# Autodesk Inventor assembly: ProbeHead - Assembly
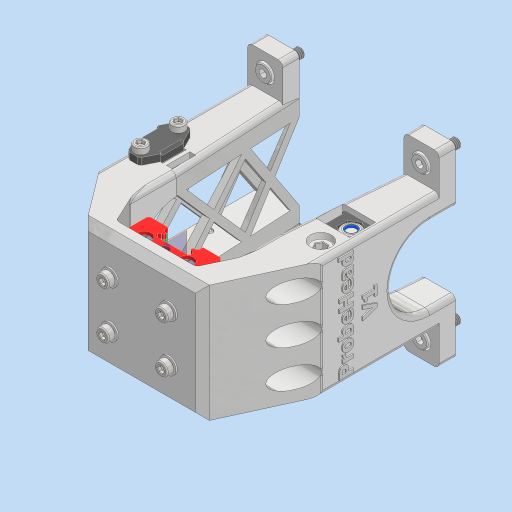
[picture p0: Inventor's stored thumbnail of the model, 512x512]
Saved by Autodesk Inventor 2023.2 (Build 272271000, 271)
## iProperties
Created: 2024-02-09
Part Number: ProbeHead - Assembly
Document SubType Name: Assembly
Designer: Nils Bade
Author: Nils Bade
## Documents named in this file (11)
- C:\Users\nilsb\Documents\Inventor\Projektarbeit-Bade\RatRig_modified\ProbeHead\ProbeHead - Assembly.iam
- C:\Users\nilsb\Documents\Inventor\Projektarbeit-Bade\RatRig_Standards\core_xy_belt_grabber v2.ipt
- C:\Users\nilsb\Documents\Inventor\Projektarbeit-Bade\RatRig_modified\MGN15 Linear-Rail-Block.ipt
- C:\Users\nilsb\Documents\Inventor\Projektarbeit-Bade\RatRig_modified\ProbeHead\ProbeHead-Arms V1.ipt
- C:\Users\nilsb\Documents\Inventor\Projektarbeit-Bade\RatRig_Standards\face_belt_grabber v2.ipt
- C:\Users\nilsb\Documents\Inventor\Projektarbeit-Bade\Schrauben\Cap Head Screw M3x12 v2.ipt
- C:\Users\nilsb\Documents\Inventor\Projektarbeit-Bade\RatRig_Standards\Hex Nut - M3 v2.ipt
- C:\Users\nilsb\Documents\Inventor\Projektarbeit-Bade\Schrauben\Cap Head Screw M5x40 v2.ipt
- C:\Users\nilsb\Documents\Inventor\Projektarbeit-Bade\RatRig_Standards\Hex Locking Nut - M5 v2.ipt
- C:\Users\nilsb\Documents\Inventor\Projektarbeit-Bade\Schrauben\Cap Head Screw M4x12 - DIN912.ipt
- C:\Users\nilsb\Documents\Inventor\Projektarbeit-Bade\Schrauben\Washer Simple M3 - DIN6902.ipt
## Components (30 placed, 10 different names)
1. ProbeHead-Arms V1:1 — Passend:1, Passend:2, Passend:3, Passend:4, Winkel:1, Winkel:2, Passend:5, Fluchtend:1, Fluchtend:2, Passend:6, Passend:8, Passend:9, Passend:11, Winkel:3, Winkel:6, Passend:24, Passend:25, Passend:26, Passend:27, Passend:28, Passend:29, Passend:30, Passend:31, Passend:36, Passend:37, Passend:38, Passend:39, Passend:40, Passend:41, Passend:42, Passend:43, Passend:44, Passend:45, Passend:46, Passend:47, Passend:48, Passend:49, Passend:50, Passend:51, Passend:52, Passend:53, Passend:54, Passend:55, Passend:60, Passend:61, Winkel:9, Winkel:10
2. core_xy_belt_grabber v2:1 — Winkel:2, Passend:5, Fluchtend:1, Winkel:7, Passend:35
3. core_xy_belt_grabber v2:2 — Passend:4, Winkel:1, Fluchtend:2, Passend:32, Passend:33, Winkel:8
4. MGN15 Linear-Rail-Block:1 — Passend:1, Passend:2, Passend:3
5. face_belt_grabber v2:1 — Passend:9, Passend:11, Passend:16, Passend:17, Passend:18, Passend:19
6. face_belt_grabber v2:2 — Passend:6, Passend:8, Passend:12, Passend:13, Passend:14, Passend:15
7. Cap Head Screw M3x12 v2:1 — Passend:16, Passend:18, Passend:20
8. Cap Head Screw M3x12 v2:2 — Passend:17, Passend:19, Passend:21, Passend:61
9. Cap Head Screw M3x12 v2:3 — Passend:12, Passend:14, Passend:22
10. Cap Head Screw M3x12 v2:4 — Passend:13, Passend:15, Passend:23, Passend:60
11. Hex Nut - M3 v2:1 — Passend:20, Winkel:3, Passend:26
12. Hex Nut - M3 v2:2 — Passend:23, Passend:25, Winkel:9
13. Hex Nut - M3 v2:3 — Passend:22, Winkel:6, Passend:24
14. Hex Nut - M3 v2:4 — Passend:21, Passend:27, Winkel:10
15. Cap Head Screw M5x40 v2:1 — Passend:29, Passend:30, Passend:34
16. Cap Head Screw M5x40 v2:2 — Passend:28, Passend:31
17. Hex Locking Nut - M5 v2:1 — Passend:32, Passend:33, Winkel:8
18. Hex Locking Nut - M5 v2:2 — Passend:34, Winkel:7, Passend:35
19. Cap Head Screw M4x12 - DIN912:1 — Passend:36, Passend:40
20. Cap Head Screw M4x12 - DIN912:2 — Passend:37, Passend:41
21. Cap Head Screw M4x12 - DIN912:3 — Passend:39, Passend:43
22. Cap Head Screw M4x12 - DIN912:4 — Passend:38, Passend:42
23. Washer Simple M3 - DIN6902:1 — Passend:44, Passend:50, Passend:59
24. Washer Simple M3 - DIN6902:2 — Passend:45, Passend:49, Passend:56
25. Washer Simple M3 - DIN6902:3 — Passend:46, Passend:51, Passend:58
26. Washer Simple M3 - DIN6902:4 — Passend:47, Passend:48, Passend:57
27. Cap Head Screw M3x12 v2:5 — Passend:52, Passend:59
28. Cap Head Screw M3x12 v2:6 — Passend:53, Passend:58
29. Cap Head Screw M3x12 v2:7 — Passend:54, Passend:56
30. Cap Head Screw M3x12 v2:8 — Passend:55, Passend:57
## Relationships (69: Mate 59, Angle 8, Flush 2)
- Passend:1 [Mate]: ProbeHead-Arms V1:1 ↔ MGN15 Linear-Rail-Block:1
- Passend:2 [Mate]: ProbeHead-Arms V1:1 ↔ MGN15 Linear-Rail-Block:1
- Passend:3 [Mate]: ProbeHead-Arms V1:1 ↔ MGN15 Linear-Rail-Block:1
- Passend:4 [Mate]: ProbeHead-Arms V1:1 ↔ core_xy_belt_grabber v2:2
- Winkel:1 [Angle] (0 deg): ProbeHead-Arms V1:1 ↔ core_xy_belt_grabber v2:2
- Winkel:2 [Angle] (0 deg): ProbeHead-Arms V1:1 ↔ core_xy_belt_grabber v2:1
- Passend:5 [Mate]: ProbeHead-Arms V1:1 ↔ core_xy_belt_grabber v2:1
- Fluchtend:1 [Flush] (2 mm): ProbeHead-Arms V1:1 ↔ core_xy_belt_grabber v2:1
- Fluchtend:2 [Flush] (2 mm): ProbeHead-Arms V1:1 ↔ core_xy_belt_grabber v2:2
- Passend:6 [Mate]: ProbeHead-Arms V1:1 ↔ face_belt_grabber v2:2
- Passend:8 [Mate]: ProbeHead-Arms V1:1 ↔ face_belt_grabber v2:2
- Passend:9 [Mate]: ProbeHead-Arms V1:1 ↔ face_belt_grabber v2:1
- Passend:11 [Mate]: ProbeHead-Arms V1:1 ↔ face_belt_grabber v2:1
- Passend:12 [Mate]: face_belt_grabber v2:2 ↔ Cap Head Screw M3x12 v2:3
- Passend:13 [Mate]: face_belt_grabber v2:2 ↔ Cap Head Screw M3x12 v2:4
- Passend:14 [Mate]: face_belt_grabber v2:2 ↔ Cap Head Screw M3x12 v2:3
- Passend:15 [Mate]: face_belt_grabber v2:2 ↔ Cap Head Screw M3x12 v2:4
- Passend:16 [Mate]: face_belt_grabber v2:1 ↔ Cap Head Screw M3x12 v2:1
- Passend:17 [Mate]: face_belt_grabber v2:1 ↔ Cap Head Screw M3x12 v2:2
- Passend:18 [Mate]: face_belt_grabber v2:1 ↔ Cap Head Screw M3x12 v2:1
- Passend:19 [Mate]: face_belt_grabber v2:1 ↔ Cap Head Screw M3x12 v2:2
- Passend:20 [Mate]: Cap Head Screw M3x12 v2:1 ↔ Hex Nut - M3 v2:1
- Passend:21 [Mate]: Cap Head Screw M3x12 v2:2 ↔ Hex Nut - M3 v2:4
- Passend:22 [Mate]: Cap Head Screw M3x12 v2:3 ↔ Hex Nut - M3 v2:3
- Passend:23 [Mate]: Cap Head Screw M3x12 v2:4 ↔ Hex Nut - M3 v2:2
- Winkel:3 [Angle] (0 deg): ProbeHead-Arms V1:1 ↔ Hex Nut - M3 v2:1
- Winkel:6 [Angle] (0 deg): ProbeHead-Arms V1:1 ↔ Hex Nut - M3 v2:3
- Passend:24 [Mate]: ProbeHead-Arms V1:1 ↔ Hex Nut - M3 v2:3
- Passend:25 [Mate]: ProbeHead-Arms V1:1 ↔ Hex Nut - M3 v2:2
- Passend:26 [Mate]: ProbeHead-Arms V1:1 ↔ Hex Nut - M3 v2:1
- Passend:27 [Mate]: ProbeHead-Arms V1:1 ↔ Hex Nut - M3 v2:4
- Passend:28 [Mate]: ProbeHead-Arms V1:1 ↔ Cap Head Screw M5x40 v2:2
- Passend:29 [Mate]: ProbeHead-Arms V1:1 ↔ Cap Head Screw M5x40 v2:1
- Passend:30 [Mate]: ProbeHead-Arms V1:1 ↔ Cap Head Screw M5x40 v2:1
- Passend:31 [Mate]: ProbeHead-Arms V1:1 ↔ Cap Head Screw M5x40 v2:2
- Passend:32 [Mate]: core_xy_belt_grabber v2:2 ↔ Hex Locking Nut - M5 v2:1
- Passend:33 [Mate]: core_xy_belt_grabber v2:2 ↔ Hex Locking Nut - M5 v2:1
- Passend:34 [Mate]: Cap Head Screw M5x40 v2:1 ↔ Hex Locking Nut - M5 v2:2
- Winkel:7 [Angle] (0 deg): core_xy_belt_grabber v2:1 ↔ Hex Locking Nut - M5 v2:2
- Passend:35 [Mate]: core_xy_belt_grabber v2:1 ↔ Hex Locking Nut - M5 v2:2
- Winkel:8 [Angle] (0 deg): core_xy_belt_grabber v2:2 ↔ Hex Locking Nut - M5 v2:1
- Passend:36 [Mate]: ProbeHead-Arms V1:1 ↔ Cap Head Screw M4x12 - DIN912:1
- Passend:37 [Mate]: ProbeHead-Arms V1:1 ↔ Cap Head Screw M4x12 - DIN912:2
- Passend:38 [Mate]: ProbeHead-Arms V1:1 ↔ Cap Head Screw M4x12 - DIN912:4
- Passend:39 [Mate]: ProbeHead-Arms V1:1 ↔ Cap Head Screw M4x12 - DIN912:3
- Passend:40 [Mate]: ProbeHead-Arms V1:1 ↔ Cap Head Screw M4x12 - DIN912:1
- Passend:41 [Mate]: ProbeHead-Arms V1:1 ↔ Cap Head Screw M4x12 - DIN912:2
- Passend:42 [Mate]: ProbeHead-Arms V1:1 ↔ Cap Head Screw M4x12 - DIN912:4
- Passend:43 [Mate]: ProbeHead-Arms V1:1 ↔ Cap Head Screw M4x12 - DIN912:3
- Passend:44 [Mate]: ProbeHead-Arms V1:1 ↔ Washer Simple M3 - DIN6902:1
- Passend:45 [Mate]: ProbeHead-Arms V1:1 ↔ Washer Simple M3 - DIN6902:2
- Passend:46 [Mate]: ProbeHead-Arms V1:1 ↔ Washer Simple M3 - DIN6902:3
- Passend:47 [Mate]: ProbeHead-Arms V1:1 ↔ Washer Simple M3 - DIN6902:4
- Passend:48 [Mate]: ProbeHead-Arms V1:1 ↔ Washer Simple M3 - DIN6902:4
- Passend:49 [Mate]: ProbeHead-Arms V1:1 ↔ Washer Simple M3 - DIN6902:2
- Passend:50 [Mate]: ProbeHead-Arms V1:1 ↔ Washer Simple M3 - DIN6902:1
- Passend:51 [Mate]: ProbeHead-Arms V1:1 ↔ Washer Simple M3 - DIN6902:3
- Passend:52 [Mate]: ProbeHead-Arms V1:1 ↔ Cap Head Screw M3x12 v2:5
- Passend:53 [Mate]: ProbeHead-Arms V1:1 ↔ Cap Head Screw M3x12 v2:6
- Passend:54 [Mate]: ProbeHead-Arms V1:1 ↔ Cap Head Screw M3x12 v2:7
- Passend:55 [Mate]: ProbeHead-Arms V1:1 ↔ Cap Head Screw M3x12 v2:8
- Passend:56 [Mate]: Washer Simple M3 - DIN6902:2 ↔ Cap Head Screw M3x12 v2:7
- Passend:57 [Mate]: Washer Simple M3 - DIN6902:4 ↔ Cap Head Screw M3x12 v2:8
- Passend:58 [Mate]: Washer Simple M3 - DIN6902:3 ↔ Cap Head Screw M3x12 v2:6
- Passend:59 [Mate]: Washer Simple M3 - DIN6902:1 ↔ Cap Head Screw M3x12 v2:5
- Passend:60 [Mate]: ProbeHead-Arms V1:1 ↔ Cap Head Screw M3x12 v2:4
- Passend:61 [Mate]: ProbeHead-Arms V1:1 ↔ Cap Head Screw M3x12 v2:2
- Winkel:9 [Angle] (0 deg): ProbeHead-Arms V1:1 ↔ Hex Nut - M3 v2:2
- Winkel:10 [Angle] (0 deg): ProbeHead-Arms V1:1 ↔ Hex Nut - M3 v2:4
